# Autodesk Inventor assembly: Rafix S20
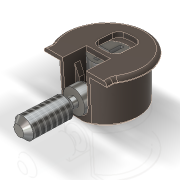
[picture p0: Inventor's stored thumbnail of the model, 180x180]
Saved by Autodesk Inventor 2024 (Build 280153000, 153)
## iProperties
RuleStatus: InUse
Created: 2023-03-20
Part Number: Rafix S20
Document SubType Name: Assembly
Designer: sauliusd
Author: sauliusd
## Documents named in this file (3)
- C:\W4INV 2024 Design\SMART HARDWARE\Rafix\Rafix S20.iam
- C:\W4INV 2024 Design\SMART HARDWARE\Rafix\Parts\Rafix Skeleton.ipt
- C:\W4INV 2024 Design\PROJECTS\MODEL STATE LIBRARY COMPONENTS\Rafix S20\Rafix.iam
## Components (3 placed, 3 different names)
1. @Skeleton — Flush:1, Flush:2, Flush:3, Insert:1
2. Rafix S20 [sub-assembly] — Insert:1, Angle:1
3. Rafix:2 [sub-assembly]
## Component patterns: (2 elements, first: Rafix S20)
## Relationships (5: Flush 3, Insert 1, Angle 1)
- Flush:1: @Skeleton
- Flush:2: @Skeleton
- Flush:3: @Skeleton
- Insert:1: @Skeleton ↔ Rafix S20
- Angle:1 (0 deg): Rafix S20
## Named parameters: ContactPatchLength = 300 mm, ContactPatchWidth = 16 mm, Offset1 = 60 mm, Offset2 = 60 mm, MaxDistance = 500 mm, YCoord = 9.5 mm, NestledBoardT = 18 mm, PillarBoardT = 16 mm, ConnectionAngle = 90 deg, Gap = 0 mm
